# Autodesk Inventor assembly: !conveyer_box
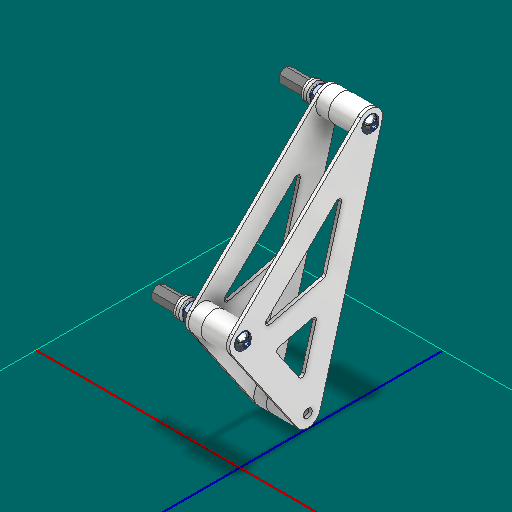
[picture p0: Inventor's stored thumbnail of the model, 512x512]
Saved by Autodesk Inventor 2025 (Build 290162000, 162)
## iProperties
Created: 2024-08-19
Part Number: !conveyer_box
Document SubType Name: Assembly
Designer: averey
Author: averey
## Documents named in this file (14)
- C:\Users\avere\vex_robotics_high_stakes\hardware\cad\ATLAS\tower\conveyer_box\structure.iam
- structure.iam
- C:\Users\avere\vex_robotics_high_stakes\hardware\cad\ATLAS\tower\conveyer_box\custom_parts\gusset.ipt
- C:\Users\avere\vex_robotics_high_stakes\hardware\cad\VEX-CAD-Inventor\Motion\Spacers\Spacer Nylon .500 OD\NSpacer White .500 OD x .250.ipt
- C:\Users\avere\vex_robotics_high_stakes\hardware\cad\VEX-CAD-Inventor\Motion\Spacers\Spacer Nylon .500 OD.ipt
- C:\Users\avere\vex_robotics_high_stakes\hardware\cad\VEX-CAD-Inventor\Motion\Spacers\Spacer Nylon .500 OD\NSpacer White .500 OD x .500.ipt
- C:\Users\avere\vex_robotics_high_stakes\hardware\cad\VEX-CAD-Inventor\Structure\Hardware\Nut Thin Nylock.ipt
- C:\Users\avere\vex_robotics_high_stakes\hardware\cad\VEX-CAD-Inventor\Motion\Spacers\Washer Teflon\TWasher .375 OD x .04000.ipt
- C:\Users\avere\vex_robotics_high_stakes\hardware\cad\VEX-CAD-Inventor\Motion\Spacers\Washer Teflon.ipt
- C:\Users\avere\vex_robotics_high_stakes\hardware\cad\VEX-CAD-Inventor\Structure\Standoff.ipt
- C:\Users\avere\vex_robotics_high_stakes\hardware\cad\VEX-CAD-Inventor\Structure\Hardware\Screw Steel - Star.ipt
- C:\Users\avere\vex_robotics_high_stakes\hardware\cad\VEX-CAD-Inventor\Structure\Standoff\Standoff .50.ipt
- C:\Users\avere\vex_robotics_high_stakes\hardware\cad\VEX-CAD-Inventor\Motion\Spacers\Washer Teflon\TWasher .375 OD x .06250.ipt
- C:\Users\avere\vex_robotics_high_stakes\hardware\cad\VEX-CAD-Inventor\Structure\Hardware\Screw Steel - Star\SScrew Star Smooth 1.250.ipt
## Components (18 placed, 8 different names)
1. gusset:1 — Insert:1, Insert:8, Insert:9
2. gusset:2 — Mate:2, Insert:1, Insert:5, Insert:6, Insert:7, Insert:27, Insert:28
3. NSpacer White .500 OD x .250:1 — Insert:4
4. NSpacer White .500 OD x .500:2 — Insert:4, Insert:6
5. NSpacer White .500 OD x .250:3 — Insert:3
6. NSpacer White .500 OD x .500:4 — Insert:3, Insert:7
7. NSpacer White .500 OD x .250:5 — Insert:2
8. NSpacer White .500 OD x .500:6 — Insert:2, Insert:5
9. Nut Thin Nylock:1 — Insert:8, Insert:26
10. Nut Thin Nylock:2 — Insert:9, Insert:23
11. Standoff .50:2 — Insert:22
12. TWasher .375 OD x .04000:2 — Insert:21, Insert:22
13. TWasher .375 OD x .06250:3 — Insert:21, Insert:23
14. Standoff .50:3
15. TWasher .375 OD x .04000:4
16. TWasher .375 OD x .06250:5 — Insert:26
17. SScrew Star Smooth 1.250:1 — Insert:28
18. SScrew Star Smooth 1.250:2 — Insert:27
## Relationships (19: Insert 17, Mate 2)
- [Mate]: gusset:1 ↔ gusset:2
- Mate:2: gusset:2
- Insert:1 (19.05 mm): gusset:1 ↔ gusset:2
- Insert:2: NSpacer White .500 OD x .250:5 ↔ NSpacer White .500 OD x .500:6
- Insert:3: NSpacer White .500 OD x .250:3 ↔ NSpacer White .500 OD x .500:4
- Insert:4: NSpacer White .500 OD x .250:1 ↔ NSpacer White .500 OD x .500:2
- Insert:5: gusset:2 ↔ NSpacer White .500 OD x .500:6
- Insert:6: gusset:2 ↔ NSpacer White .500 OD x .500:2
- Insert:7: gusset:2 ↔ NSpacer White .500 OD x .500:4
- Insert:8: gusset:1 ↔ Nut Thin Nylock:1
- Insert:9: gusset:1 ↔ Nut Thin Nylock:2
- Insert:21: TWasher .375 OD x .04000:2 ↔ TWasher .375 OD x .06250:3
- Insert:22: Standoff .50:2 ↔ TWasher .375 OD x .04000:2
- Insert:23: Nut Thin Nylock:2 ↔ TWasher .375 OD x .06250:3
- [Insert]: TWasher .375 OD x .04000:4 ↔ TWasher .375 OD x .06250:5
- [Insert]: Standoff .50:3 ↔ TWasher .375 OD x .04000:4
- Insert:26: Nut Thin Nylock:1 ↔ TWasher .375 OD x .06250:5
- Insert:27: gusset:2 ↔ SScrew Star Smooth 1.250:2
- Insert:28: gusset:2 ↔ SScrew Star Smooth 1.250:1
## Named parameters: d33_d30 = 0 mm, d34_d31 = 0 mm
